# Autodesk Inventor assembly: 飞控外壳
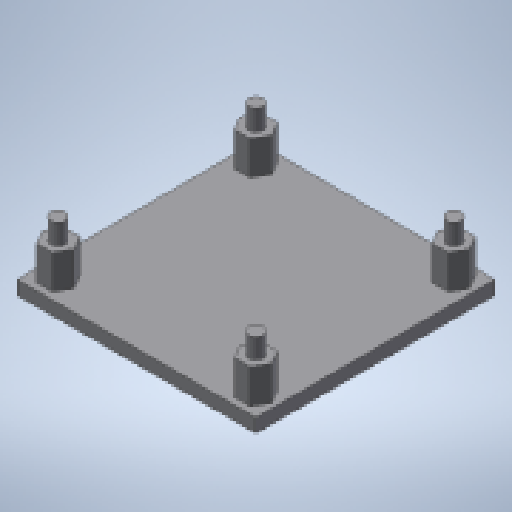
[picture p0: Inventor's stored thumbnail of the model, 512x512]
Saved by Autodesk Inventor 2025.2 (Build 292293000, 293)
## iProperties
Created: 2026-04-16
Part Number: 飞控外壳
Document SubType Name: Assembly
Designer: BO‘S_SLAVE
Author: BO‘S_SLAVE
## Documents named in this file (3)
- D:\UAV\esp drone\diy-drone\mechanical\新版 4.5\飞控盒\飞控盒.iam
- D:\UAV\esp drone\diy-drone\mechanical\新版 4.5\飞控盒\飞控外壳.ipt
- D:\UAV\esp drone\diy-drone\mechanical\新版 4.5\飞控盒\铜柱.ipt
## Components (5 placed, 2 different names)
1. 飞控外壳:1 — 表面齐平:1, 配合:1, 配合:2, 配合:3, 配合:4, 配合:5, 配合:6, 配合:7
2. 铜柱:1 — 表面齐平:1, 配合:1
3. 铜柱:2 — 配合:2, 配合:7
4. 铜柱:3 — 配合:3, 配合:6, 表面齐平:2
5. 铜柱:4 — 配合:4, 配合:5, 表面齐平:2
## Relationships (9: Mate 7, Flush 2)
- 表面齐平:1 [Flush]: 飞控外壳:1 ↔ 铜柱:1
- 配合:1 [Mate]: 飞控外壳:1 ↔ 铜柱:1
- 配合:2 [Mate]: 飞控外壳:1 ↔ 铜柱:2
- 配合:3 [Mate]: 飞控外壳:1 ↔ 铜柱:3
- 配合:4 [Mate]: 飞控外壳:1 ↔ 铜柱:4
- 配合:5 [Mate]: 飞控外壳:1 ↔ 铜柱:4
- 配合:6 [Mate]: 飞控外壳:1 ↔ 铜柱:3
- 配合:7 [Mate]: 飞控外壳:1 ↔ 铜柱:2
- 表面齐平:2 [Flush]: 铜柱:3 ↔ 铜柱:4
